# Autodesk Inventor assembly: SnowBlowerMotorAndHub
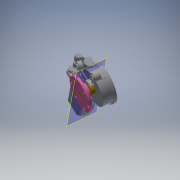
[picture p0: Inventor's stored thumbnail of the model, 180x180]
Saved by Autodesk Inventor 2016 SP1 (Build 200210100, 210)
## iProperties
Created: 2016-01-24
Part Number: SnowBlowerMotorAndHub
Document SubType Name: Assembly
Designer: steele
Author: steele
## Documents named in this file (3)
- C:\snobotics\CAD-Development\robSteele\SnoBotics2016\AM Parts\SnowBlowerMotorAndHub.iam
- C:\snobotics\CAD-Development\robSteele\SnoBotics2016\AM Parts\AM-2235-snow-blower.iam
- C:\snobotics\CAD-Development\robSteele\SnoBotics2016\AM Parts\am-2279+10mm+DD+Bore+Hub-snow-blower.ipt
## Components (2 placed, 2 different names)
1. AM-2235-snow-blower:1 [sub-assembly] — Flush:1, Mate:1
2. am-2279+10mm+DD+Bore+Hub-snow-blower:1 — Flush:1, Mate:1
## Relationships (2: Flush 1, Mate 1)
- Flush:1: AM-2235-snow-blower:1 ↔ am-2279+10mm+DD+Bore+Hub-snow-blower:1
- Mate:1: AM-2235-snow-blower:1 ↔ am-2279+10mm+DD+Bore+Hub-snow-blower:1
